# Autodesk Inventor assembly: small base wheel
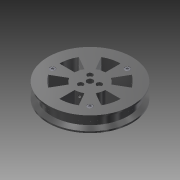
[picture p0: Inventor's stored thumbnail of the model, 180x180]
Saved by Autodesk Inventor 2011 (Build 150239000, 239)
## iProperties
Created: 2010-04-19
Part Number: small base wheel
Document SubType Name: Assembly
Designer: lucio
Author: lucio
## Documents named in this file (4)
- C:\Users\lucio\Documents\Inventor\caterpillar\small base wheel.iam
- C:\Users\lucio\Documents\Inventor\caterpillar\wheel small.ipt
- C:\Users\lucio\Documents\Inventor\Content Center Files\R2011\en-US\ANSI B18.3.1M(3)\ANSI B18.3.1M - M4x0.7 x 16(5).ipt
- C:\Users\lucio\Documents\Inventor\Content Center Files\R2011\en-US\ANSI B 18.2.4.1 M(1)\ANSI B 18.2.4.1 M - M4 x 0.7Style 2.ipt
## Components (8 placed, 3 different names)
1. wheel small:1 — Mate:1, Mate:2, Mate:3, Insert:4, Insert:5, Insert:6
2. wheel small:2 — Mate:1, Mate:2, Mate:3, Insert:1, Insert:2, Insert:3
3. Drilled Broached Hexagon Socket Head Cap Screw - 6 Holes - Metric M4x0.7 x 16:1 — Insert:2
4. Drilled Broached Hexagon Socket Head Cap Screw - 6 Holes - Metric M4x0.7 x 16:2 — Insert:3
5. Drilled Broached Hexagon Socket Head Cap Screw - 6 Holes - Metric M4x0.7 x 16:3 — Insert:1
6. Hex Nut Metric M4 x 0.7:1 — Insert:4
7. Hex Nut Metric M4 x 0.7:2 — Insert:5
8. Hex Nut Metric M4 x 0.7:3 — Insert:6
## Relationships (9: Insert 6, Mate 3)
- Mate:1: wheel small:1 ↔ wheel small:2
- Mate:2: wheel small:1 ↔ wheel small:2
- Mate:3: wheel small:1 ↔ wheel small:2
- Insert:1: wheel small:2 ↔ Drilled Broached Hexagon Socket Head Cap Screw - 6 Holes - Metric M4x0.7 x 16:3
- Insert:2: wheel small:2 ↔ Drilled Broached Hexagon Socket Head Cap Screw - 6 Holes - Metric M4x0.7 x 16:1
- Insert:3: wheel small:2 ↔ Drilled Broached Hexagon Socket Head Cap Screw - 6 Holes - Metric M4x0.7 x 16:2
- Insert:4: wheel small:1 ↔ Hex Nut Metric M4 x 0.7:1
- Insert:5: wheel small:1 ↔ Hex Nut Metric M4 x 0.7:2
- Insert:6: wheel small:1 ↔ Hex Nut Metric M4 x 0.7:3
